# Autodesk Inventor assembly: Tornillo Molienda
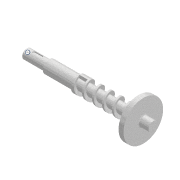
[picture p0: Inventor's stored thumbnail of the model, 180x180]
Saved by Autodesk Inventor 2021 (Build 250183000, 183)
## iProperties
Created: 2022-02-07
Part Number: Tornillo Molienda
Document SubType Name: Assembly
Designer: Santiago
Mass: 402.845 g
Surface Area: 362.523 cm^2
Volume: 149.202 cm^3
Density: 2.7 g/cm^3
Author: Santiago
## Documents named in this file (2)
- C:\Users\user\Desktop\Ingeniería Mecánica UN\7. Séptimo Semestre\Diseño de Elementos de Máquinas 1\Proyecto Moledora\Tornillo Molienda.iam
- C:\Users\user\Desktop\Ingeniería Mecánica UN\7. Séptimo Semestre\Diseño de Elementos de Máquinas 1\Proyecto Moledora\Shaft1.ipt
## Components (1 placed, 1 different names)
1. Shaft:1 — Tangent:1, Tangent:2
## Relationships (5: Angle 2, Tangent 2, Flush 1)
- Angle:1 (0 deg)
- Tangent:1: Shaft:1
- Angle:2 (0 deg)
- Tangent:2: Shaft:1
- Flush:1 (-40 mm)
